# Autodesk Inventor assembly: Assembly1
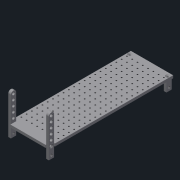
[picture p0: Inventor's stored thumbnail of the model, 180x180]
Saved by Autodesk Inventor 2021.1 (Build 251245000, 245)
## iProperties
Created: 2020-05-07
Part Number: Assembly1
Document SubType Name: Assembly
Designer: Workshop Tech
Author: Workshop Tech
## Documents named in this file (4)
- C:\Users\bestm\Desktop\End of Dec Work\Mounting Platform\Mounting Platform.iam
- C:\Users\bestm\Desktop\End of Dec Work\Mounting Platform\Mounting plate.ipt
- C:\Users\bestm\Desktop\End of Dec Work\Mounting Platform\Rear Leg.ipt
- C:\Users\bestm\Desktop\End of Dec Work\Mounting Platform\Pivot Leg.ipt
## Components (5 placed, 3 different names)
1. Mounting plate:1 — Mate:6, Mate:8, Mate:9, Angle:1, Mate:10, Angle:2, Mate:11, Angle:3, Mate:12, Mate:13, Mate:14, Angle:4
2. Rear Leg:1 — Mate:8, Mate:9, Angle:1
3. Rear Leg:2 — Mate:6, Mate:10, Angle:2
4. Pivot Leg:5 — Mate:13, Mate:14, Angle:4
5. Pivot Leg:6 — Mate:11, Angle:3, Mate:12
## Relationships (12: Mate 8, Angle 4)
- Mate:6: Mounting plate:1 ↔ Rear Leg:2
- Mate:8: Mounting plate:1 ↔ Rear Leg:1
- Mate:9: Mounting plate:1 ↔ Rear Leg:1
- Angle:1 (0 deg): Mounting plate:1 ↔ Rear Leg:1
- Mate:10: Mounting plate:1 ↔ Rear Leg:2
- Angle:2 (0 deg): Mounting plate:1 ↔ Rear Leg:2
- Mate:11: Mounting plate:1 ↔ Pivot Leg:6
- Angle:3 (0 deg): Mounting plate:1 ↔ Pivot Leg:6
- Mate:12: Mounting plate:1 ↔ Pivot Leg:6
- Mate:13: Mounting plate:1 ↔ Pivot Leg:5
- Mate:14: Mounting plate:1 ↔ Pivot Leg:5
- Angle:4 (0 deg): Mounting plate:1 ↔ Pivot Leg:5
